# Autodesk Inventor assembly: smart servo with servo block
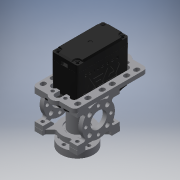
[picture p0: Inventor's stored thumbnail of the model, 180x180]
Saved by Autodesk Inventor 2019 (Build 230136000, 136)
## iProperties
Created: 2018-10-02
Part Number: smart servo with servo block
Document SubType Name: Assembly
Designer: User
Author: User
## Documents named in this file (6)
- C:\Robotics\CAD\2018-19_CAD\smart servo with servo block.iam
- C:\Robotics\CAD\COTSParts\Rev\REV-41-1097SmartServo.ipt
- C:\Robotics\CAD\COTSParts\Actobotics\637 parts\637110ServoBlock24THubShaft\575112.ipt
- C:\Robotics\CAD\COTSParts\Actobotics\637 parts\637110ServoBlock24THubShaft\525122.ipt
- C:\Robotics\CAD\COTSParts\Actobotics\637 parts\637110ServoBlock24THubShaft\535118 assembly.ipt
- C:\Robotics\CAD\COTSParts\Actobotics\637 parts\637110ServoBlock24THubShaft\545420.ipt
## Components (6 placed, 5 different names)
1. REV-41-1097SmartServo:1 — Mate:9, Insert:1, Mate:10, Angle:3
2. 575112:1 — Mate:2, Angle:1, Mate:3, Mate:10, Angle:3
3. 525122:1 — Mate:8, Mate:9, Insert:1
4. 535118 assembly:1 — Mate:5, Mate:8, Mate:11, Mate:12, Mate:13, Mate:14
5. 545420:1 — Mate:2, Angle:1, Mate:5, Mate:13, Mate:14
6. 545420:2 — Mate:3, Mate:11, Mate:12
## Relationships (13: Mate 10, Angle 2, Insert 1)
- Mate:2: 575112:1 ↔ 545420:1
- Angle:1 (0 deg): 575112:1 ↔ 545420:1
- Mate:3: 575112:1 ↔ 545420:2
- Mate:5: 535118 assembly:1 ↔ 545420:1
- Mate:8: 525122:1 ↔ 535118 assembly:1
- Mate:9: REV-41-1097SmartServo:1 ↔ 525122:1
- Insert:1: REV-41-1097SmartServo:1 ↔ 525122:1
- Mate:10: REV-41-1097SmartServo:1 ↔ 575112:1
- Angle:3 (0 deg): REV-41-1097SmartServo:1 ↔ 575112:1
- Mate:11: 535118 assembly:1 ↔ 545420:2
- Mate:12: 535118 assembly:1 ↔ 545420:2
- Mate:13: 535118 assembly:1 ↔ 545420:1
- Mate:14: 535118 assembly:1 ↔ 545420:1
